# Autodesk Inventor assembly: Naroznik
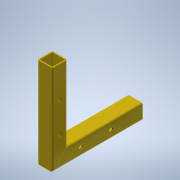
[picture p0: Inventor's stored thumbnail of the model, 180x180]
Saved by Autodesk Inventor 2021 (Build 250183000, 183)
## iProperties
Created: 2024-04-18
Part Number: Naroznik
Document SubType Name: Assembly
Designer: Michal
Author: Michal
## Documents named in this file (3)
- C:\Users\Michal\Documents\GitHub\PNW_PhotoBoothFrame_3D\Naroznik.iam
- C:\Users\Michal\Documents\GitHub\PNW_PhotoBoothFrame_3D\narrow high rectangular\beam 25x25x2 2-1.ipt
- C:\Users\Michal\Documents\GitHub\PNW_PhotoBoothFrame_3D\Naroznik profil 1.ipt
## Components (2 placed, 2 different names)
1. beam 25x25x2 2-1:1 — Mate:1, Flush:1, Mate:2
2. Naroznik profil 1:1 — Mate:1, Flush:1, Mate:2
## Relationships (3: Mate 2, Flush 1)
- Mate:1: beam 25x25x2 2-1:1 ↔ Naroznik profil 1:1
- Flush:1: beam 25x25x2 2-1:1 ↔ Naroznik profil 1:1
- Mate:2: beam 25x25x2 2-1:1 ↔ Naroznik profil 1:1
